# Autodesk Inventor assembly: Сборка_Датчик
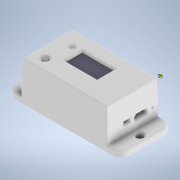
[picture p0: Inventor's stored thumbnail of the model, 180x180]
Saved by Autodesk Inventor 2022 (Build 260153000, 153)
## iProperties
Created: 2022-01-08
Part Number: Сборка_Датчик
Document SubType Name: Assembly
Designer: Me
Author: Me
## Documents named in this file (4)
- D:\my_projects\Curse\3D\Сборка\Сборка_Датчик.iam
- D:\my_projects\Curse\3D\Сборка\case_down.ipt
- D:\my_projects\Curse\3D\Сборка\case_up.ipt
- D:\my_projects\Curse\3D\Сборка\Curse_PCB.iam
## Components (3 placed, 3 different names)
1. case_down:1 — Совмещение:4, Совмещение:5, Совмещение:6, Вставка:1
2. case_up:1 — Совмещение:4, Совмещение:5, Совмещение:6
3. Curse_PCB:1 [sub-assembly] — Вставка:1
## Relationships (4: Mate 3, Insert 1)
- Совмещение:4 [Mate]: case_down:1 ↔ case_up:1
- Совмещение:5 [Mate] (1 mm): case_down:1 ↔ case_up:1
- Совмещение:6 [Mate] (1 mm): case_down:1 ↔ case_up:1
- Вставка:1 [Insert]: case_down:1 ↔ Curse_PCB:1
